# Autodesk Inventor assembly: 000200
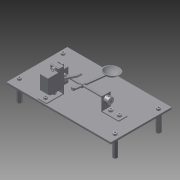
[picture p0: Inventor's stored thumbnail of the model, 180x180]
Saved by Autodesk Inventor 2015 (Build 190159000, 159)
## iProperties
Created: 2015-05-29
Part Number: 000200
Document SubType Name: Assembly
Designer: Wesley
Author: Wesley
## Documents named in this file (13)
- C:\Users\cm7078\Desktop\EngineeringFinal\Engineering\Engineering Documentation\0002__\000200.iam
- C:\Users\cm7078\Desktop\EngineeringFinal\Engineering\Engineering Documentation\0002__\000201.ipt
- C:\Users\cm7078\Desktop\EngineeringFinal\Engineering\Engineering Documentation\0002__\000204.ipt
- C:\Users\cm7078\Desktop\EngineeringFinal\Engineering\Engineering Documentation\0002__\000203.ipt
- C:\Users\cm7078\Desktop\EngineeringFinal\Engineering\Engineering Documentation\0002__\000205.ipt
- C:\Users\cm7078\Desktop\EngineeringFinal\Engineering\Engineering Documentation\0002__\000208.ipt
- C:\Users\cm7078\Desktop\EngineeringFinal\Engineering\Engineering Documentation\0002__\000206.ipt
- C:\Users\cm7078\Desktop\EngineeringFinal\Engineering\Engineering Documentation\0002__\000207.ipt
- C:\Users\cm7078\Desktop\EngineeringFinal\Engineering\Engineering Documentation\0002__\000209.ipt
- C:\Users\cm7078\Desktop\EngineeringFinal\Engineering\Engineering Documentation\0002__\000210-1.ipt
- C:\Users\cm7078\Desktop\EngineeringFinal\Engineering\Engineering Documentation\0001__\000106.ipt
- C:\Users\cm7078\Desktop\EngineeringFinal\Engineering\Engineering Documentation\0002__\000202.ipt
- C:\Users\cm7078\Desktop\EngineeringFinal\Engineering\Engineering Documentation\0002__\000210-2.ipt
## Components (32 placed, 12 different names)
1. 000201:1 — Mate:1, Mate:2, Mate:3, Mate:4, Mate:5, Mate:6, Mate:7, Mate:8, Mate:9, Mate:13, Mate:14, Mate:15, Mate:28, Mate:32, Mate:37, Mate:38, Mate:41, Mate:42, Mate:43, Mate:44, Mate:45, Mate:46, Mate:47, Mate:48, Mate:49, Mate:50, Mate:52, Mate:53, Mate:54, Mate:55, Mate:56, Mate:57, Mate:63, Mate:65
2. 000204:1 — Mate:4, Mate:5, Mate:6, Mate:24, Mate:25, Mate:26, Mate:29, Mate:33
3. 000204:2 — Mate:7, Mate:8, Mate:9, Mate:10, Mate:12, Flush:1, Mate:22, Mate:34, Mate:35, Mate:39
4. 000203:1 — Mate:10, Mate:11, Flush:1, Mate:21, Mate:23
5. 000205:1 — Mate:11, Mate:12
6. 000208:1 — Mate:13, Mate:14, Mate:15, Mate:16, Mate:17, Mate:19, Mate:58, Mate:59, Mate:60, Mate:61, Mate:66, Mate:69
7. 000206:1 — Mate:16, Mate:17, Mate:18, Mate:19, Mate:20, Mate:67
8. 000207:1 — Mate:18, Mate:20
9. 000209:1 — Mate:21, Mate:22
10. 000209:2 — Mate:23, Mate:24
11. 000210-1:1 — Mate:34, Mate:35, Mate:36
12. 000210-1:2 — Mate:38, Mate:39, Mate:40
13. 000210-1:3 — Mate:25, Mate:26, Mate:27
14. 000210-1:4 — Mate:29, Mate:31, Mate:33
15. 000106:1 — Mate:36, Mate:37
16. 000106:2 — Mate:40, Mate:41
17. 000106:3 — Mate:27, Mate:28
18. 000106:4 — Mate:31, Mate:32
19. 000202:1 — Mate:54, Mate:55
20. 000202:2 — Mate:42, Mate:43
21. 000202:3 — Mate:50, Mate:51, Mate:52
22. 000202:4 — Mate:46, Mate:47
23. 000210-1:5 — Mate:56, Mate:57
24. 000210-1:6 — Mate:48, Mate:49
25. 000210-1:7 — Mate:51, Mate:53
26. 000210-1:8 — Mate:44, Mate:45
27. 000106:5 — Mate:68, Mate:69
28. 000210-1:10 — Mate:60, Mate:61, Mate:64
29. 000106:6 — Mate:64, Mate:65
30. 000210-1:11 — Mate:58, Mate:59, Mate:62
31. 000106:7 — Mate:62, Mate:63
32. 000210-2:1 — Mate:66, Mate:67, Mate:68
## Relationships (69: Mate 68, Flush 1)
- Mate:1: 000201:1
- Mate:2: 000201:1
- Mate:3: 000201:1
- Mate:4: 000201:1 ↔ 000204:1
- Mate:5: 000201:1 ↔ 000204:1
- Mate:6: 000201:1 ↔ 000204:1
- Mate:7: 000201:1 ↔ 000204:2
- Mate:8: 000201:1 ↔ 000204:2
- Mate:9: 000201:1 ↔ 000204:2
- Mate:10: 000204:2 ↔ 000203:1
- Mate:11: 000203:1 ↔ 000205:1
- Mate:12 (31.75 mm): 000204:2 ↔ 000205:1
- Mate:13: 000201:1 ↔ 000208:1
- Mate:14: 000201:1 ↔ 000208:1
- Mate:15: 000201:1 ↔ 000208:1
- Mate:16: 000208:1 ↔ 000206:1
- Mate:17: 000208:1 ↔ 000206:1
- Mate:18: 000206:1 ↔ 000207:1
- Mate:19: 000208:1 ↔ 000206:1
- Mate:20 (0.254 mm): 000206:1 ↔ 000207:1
- Flush:1 (-6.35 mm): 000204:2 ↔ 000203:1
- Mate:21: 000203:1 ↔ 000209:1
- Mate:22: 000204:2 ↔ 000209:1
- Mate:23: 000203:1 ↔ 000209:2
- Mate:24: 000204:1 ↔ 000209:2
- Mate:25: 000204:1 ↔ 000210-1:3
- Mate:26: 000204:1 ↔ 000210-1:3
- Mate:27: 000210-1:3 ↔ 000106:3
- Mate:28: 000201:1 ↔ 000106:3
- Mate:29: 000204:1 ↔ 000210-1:4
- Mate:31: 000210-1:4 ↔ 000106:4
- Mate:32: 000201:1 ↔ 000106:4
- Mate:33: 000204:1 ↔ 000210-1:4
- Mate:34: 000204:2 ↔ 000210-1:1
- Mate:35: 000204:2 ↔ 000210-1:1
- Mate:36: 000210-1:1 ↔ 000106:1
- Mate:37: 000201:1 ↔ 000106:1
- Mate:38: 000201:1 ↔ 000210-1:2
- Mate:39: 000204:2 ↔ 000210-1:2
- Mate:40: 000210-1:2 ↔ 000106:2
- Mate:41: 000201:1 ↔ 000106:2
- Mate:42: 000201:1 ↔ 000202:2
- Mate:43: 000201:1 ↔ 000202:2
- Mate:44: 000201:1 ↔ 000210-1:8
- Mate:45: 000201:1 ↔ 000210-1:8
- Mate:46: 000201:1 ↔ 000202:4
- Mate:47: 000201:1 ↔ 000202:4
- Mate:48: 000201:1 ↔ 000210-1:6
- Mate:49: 000201:1 ↔ 000210-1:6
- Mate:50: 000201:1 ↔ 000202:3
- Mate:51: 000202:3 ↔ 000210-1:7
- Mate:52: 000201:1 ↔ 000202:3
- Mate:53: 000201:1 ↔ 000210-1:7
- Mate:54: 000201:1 ↔ 000202:1
- Mate:55: 000201:1 ↔ 000202:1
- Mate:56: 000201:1 ↔ 000210-1:5
- Mate:57: 000201:1 ↔ 000210-1:5
- Mate:58: 000208:1 ↔ 000210-1:11
- Mate:59: 000208:1 ↔ 000210-1:11
- Mate:60: 000208:1 ↔ 000210-1:10
- Mate:61: 000208:1 ↔ 000210-1:10
- Mate:62: 000210-1:11 ↔ 000106:7
- Mate:63: 000201:1 ↔ 000106:7
- Mate:64: 000210-1:10 ↔ 000106:6
- Mate:65: 000201:1 ↔ 000106:6
- Mate:66: 000208:1 ↔ 000210-2:1
- Mate:67: 000206:1 ↔ 000210-2:1
- Mate:68: 000106:5 ↔ 000210-2:1
- Mate:69: 000208:1 ↔ 000106:5
